# Autodesk Inventor assembly: CIMWithGearBox
Saved by Autodesk Inventor 2016 (Build 200138000, 138)
## iProperties
Created: 2017-01-09
Part Number: CIMWithGearBox
Document SubType Name: Assembly
Designer: Dhruv
Author: Dhruv
## Documents named in this file (3)
- C:\Users\Dhruv\Desktop\MISC\FRC 2017\supporting_parts\CIMWithGearBox.iam
- C:\Users\Dhruv\Desktop\MISC\FRC 2017\supporting_parts\am-2598_107 2016 KOP Toughbox Mini.iam
- C:\Users\Dhruv\Desktop\MISC\FRC 2017\supporting_parts\am-0255+2.5inch+CIM+Motor.ipt
## Components (3 placed, 2 different names)
1. am-2598_107 2016 KOP Toughbox Mini:1 [sub-assembly]
2. am-0255+2.5inch+CIM+Motor:1
3. am-0255+2.5inch+CIM+Motor:2
## Relationships (6: Mate 6)
- [Mate]: am-2598_107 2016 KOP Toughbox Mini:1 ↔ am-0255+2.5inch+CIM+Motor:1
- [Mate]: am-2598_107 2016 KOP Toughbox Mini:1 ↔ am-0255+2.5inch+CIM+Motor:1
- [Mate]: am-2598_107 2016 KOP Toughbox Mini:1 ↔ am-0255+2.5inch+CIM+Motor:1
- [Mate]: am-2598_107 2016 KOP Toughbox Mini:1 ↔ am-0255+2.5inch+CIM+Motor:2
- [Mate]: am-2598_107 2016 KOP Toughbox Mini:1 ↔ am-0255+2.5inch+CIM+Motor:2
- [Mate]: am-2598_107 2016 KOP Toughbox Mini:1 ↔ am-0255+2.5inch+CIM+Motor:2
